# Autodesk Inventor assembly: Nose Gear Assembly
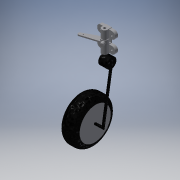
[picture p0: Inventor's stored thumbnail of the model, 180x180]
Saved by Autodesk Inventor 2018 (Build 220112000, 112)
## iProperties
Created: 2018-08-04
Part Number: Nose Gear Assembly
Document SubType Name: Assembly
Designer: Michael Gunderman
Mass: 98 g
Surface Area: 215.129 cm^2
Volume: 125.728 cm^3
Density: 0.779459 g/cm^3
Author: Michael Gunderman
## Documents named in this file (4)
- C:\Users\Michael Gunderman\Documents\Special Projects\Echo 1\CAD work\Systems\Landing Gear\Nose Gear Assembly.iam
- C:\Users\Michael Gunderman\Documents\Special Projects\Echo 1\CAD work\Systems\Landing Gear\Nose Gear Mounting Block.ipt
- C:\Users\Michael Gunderman\Documents\Special Projects\Echo 1\CAD work\Systems\Landing Gear\Nose Gear Rod and Wheel.ipt
- C:\Users\Michael Gunderman\Documents\Special Projects\Echo 1\CAD work\Systems\Landing Gear\Nose Gear Steering Arm.ipt
## Components (3 placed, 3 different names)
1. Nose Gear Mounting Block:1 — Mate:1, Mate:3
2. Nose Gear Rod and Wheel:1 — Mate:1, Mate:2
3. Nose Gear Steering Arm:1 — Mate:2, Mate:3
## Relationships (3: Mate 3)
- Mate:1: Nose Gear Mounting Block:1 ↔ Nose Gear Rod and Wheel:1
- Mate:2: Nose Gear Rod and Wheel:1 ↔ Nose Gear Steering Arm:1
- Mate:3: Nose Gear Mounting Block:1 ↔ Nose Gear Steering Arm:1
